# Autodesk Inventor assembly: CAR_000_FullCarousel
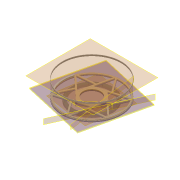
[picture p0: Inventor's stored thumbnail of the model, 180x180]
Saved by Autodesk Inventor 2020 (Build 240168000, 168)
## iProperties
Created: 2020-01-29
Part Number: CAR_000_FullCarousel
Document SubType Name: Assembly
Designer: user
Mass: 2891.81 g
Surface Area: 19758 cm^2
Volume: 2837.5 cm^3
Density: 1.01914 g/cm^3
Author: user
## Documents named in this file (4)
- C:\Users\mdill\Documents\GrabCAD\Infinite Recharge 2020\Build season\CAR_000_FullCarousel.iam
- C:\Users\mdill\Documents\GrabCAD\Infinite Recharge 2020\Build season\CAR_007_Walls.ipt
- C:\Users\mdill\Documents\GrabCAD\Infinite Recharge 2020\Build season\CAR_021_BracePattern.iam
- C:\Users\mdill\Documents\GrabCAD\Infinite Recharge 2020\Build season\CAR_022_AluminumRing.ipt
## Components (4 placed, 3 different names)
1. CAR_021_BracePattern:1 [sub-assembly] — Insert:1, Mate:1, Mate:3, Mate:4, Mate:5, Mate:6, Flush:1
2. CAR_007_Walls:1 — Insert:1, Insert:2, Insert:3
3. CAR_022_AluminumRing:1 — Insert:3
4. CAR_022_AluminumRing:2 — Insert:2
## Relationships (12: Mate 8, Insert 3, Flush 1)
- Insert:1: CAR_021_BracePattern:1 ↔ CAR_007_Walls:1
- Mate:1: CAR_021_BracePattern:1
- Mate:2
- Mate:3: CAR_021_BracePattern:1
- Mate:4: CAR_021_BracePattern:1
- Mate:5: CAR_021_BracePattern:1
- Mate:6: CAR_021_BracePattern:1
- Mate:7
- Mate:8
- Insert:2: CAR_007_Walls:1 ↔ CAR_022_AluminumRing:2
- Insert:3: CAR_007_Walls:1 ↔ CAR_022_AluminumRing:1
- Flush:1 (152.4 mm): CAR_021_BracePattern:1
